# Autodesk Inventor assembly: Version 2 mockup
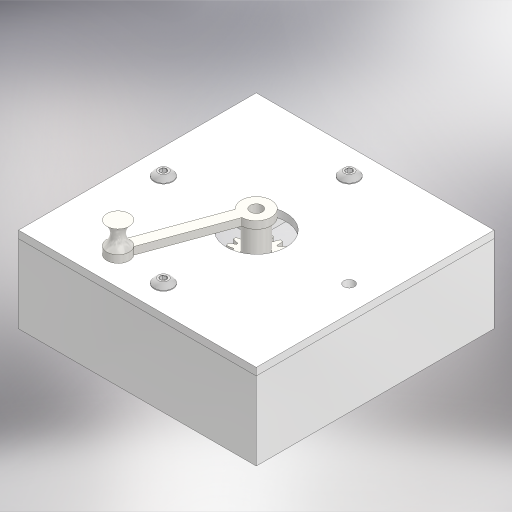
[picture p0: Inventor's stored thumbnail of the model, 512x512]
Saved by Autodesk Inventor 2024 (Build 280153000, 153)
## iProperties
Created: 2023-10-08
Part Number: Version 2 mockup
Document SubType Name: Assembly
Designer: byrne
Author: byrne
## Documents named in this file (9)
- C:\Users\byrne\OneDrive\Documents\Inventor\RAI\Fall 2023 Version\Unit.iam
- C:\Users\byrne\OneDrive\Documents\Inventor\RAI\Fall 2023 Version\Pololu#1053 v4.ipt
- C:\Users\byrne\OneDrive\Documents\Inventor\RAI\Fall 2023 Version\Dual Servo Attachment.ipt
- C:\Users\byrne\OneDrive\Documents\Inventor\RAI\Fall 2023 Version\Frame.ipt
- C:\Users\byrne\OneDrive\Documents\Inventor\RAI\Fall 2023 Version\Spur Gears1.iam
- C:\Users\byrne\OneDrive\Documents\Inventor\RAI\93365A140_Tapered Heat-Set Inserts for Plastic\93365A140_Tapered Heat-Set Inserts for Plastic.ipt
- C:\Users\byrne\OneDrive\Documents\Inventor\RAI\Fall 2023 Version\Top plate.ipt
- C:\Users\byrne\OneDrive\Documents\Inventor\RAI\98164A134_316 Stainless Steel Button Head Hex Drive Screw\98164A134_316 Stainless Steel Button Head Hex Drive Screw.ipt
- C:\Users\byrne\OneDrive\Documents\Inventor\RAI\Small Spacer for v3.ipt
## Components (12 placed, 8 different names)
1. Frame:1 — Mate:6, Mate:7, Flush:1, Mate:10, Insert:6, Insert:7, Insert:8, Insert:9, Insert:10, Insert:15
2. Pololu#1053 v4:1 — Insert:1, Mate:6, Mate:7, Flush:1, Mate:8, Angle:1
3. Dual Servo Attachment:1 — Insert:1, Mate:11, Mate:12
4. Spur Gears:1 [sub-assembly] — Mate:8, Mate:10, Mate:11, Mate:12, Angle:1, Insert:14
5. 93365A140_Tapered Heat-Set Inserts for Plastic:1 — Insert:8
6. 93365A140_Tapered Heat-Set Inserts for Plastic:2 — Insert:7
7. 93365A140_Tapered Heat-Set Inserts for Plastic:3 — Insert:6
8. Top plate:1 — Insert:9, Insert:10, Insert:11, Insert:12, Insert:13
9. 98164A134_316 Stainless Steel Button Head Hex Drive Screw:1 — Insert:13
10. 98164A134_316 Stainless Steel Button Head Hex Drive Screw:2 — Insert:12
11. 98164A134_316 Stainless Steel Button Head Hex Drive Screw:3 — Insert:11
12. Small Spacer for v3:1 — Insert:14, Insert:15
## Relationships (19: Insert 11, Mate 6, Flush 1, Angle 1)
- Insert:1: Pololu#1053 v4:1 ↔ Dual Servo Attachment:1
- Mate:6 (0.5 mm): Frame:1 ↔ Pololu#1053 v4:1
- Mate:7 (0.5 mm): Frame:1 ↔ Pololu#1053 v4:1
- Flush:1: Frame:1 ↔ Pololu#1053 v4:1
- Mate:8: Pololu#1053 v4:1 ↔ Spur Gears:1
- Mate:10: Frame:1 ↔ Spur Gears:1
- Mate:11: Dual Servo Attachment:1 ↔ Spur Gears:1
- Mate:12: Dual Servo Attachment:1 ↔ Spur Gears:1
- Angle:1 (0 deg): Pololu#1053 v4:1 ↔ Spur Gears:1
- Insert:6: Frame:1 ↔ 93365A140_Tapered Heat-Set Inserts for Plastic:3
- Insert:7: Frame:1 ↔ 93365A140_Tapered Heat-Set Inserts for Plastic:2
- Insert:8: Frame:1 ↔ 93365A140_Tapered Heat-Set Inserts for Plastic:1
- Insert:9: Frame:1 ↔ Top plate:1
- Insert:10: Frame:1 ↔ Top plate:1
- Insert:11: Top plate:1 ↔ 98164A134_316 Stainless Steel Button Head Hex Drive Screw:3
- Insert:12: Top plate:1 ↔ 98164A134_316 Stainless Steel Button Head Hex Drive Screw:2
- Insert:13: Top plate:1 ↔ 98164A134_316 Stainless Steel Button Head Hex Drive Screw:1
- Insert:14: Spur Gears:1 ↔ Small Spacer for v3:1
- Insert:15: Frame:1 ↔ Small Spacer for v3:1
